# Autodesk Inventor assembly: roka
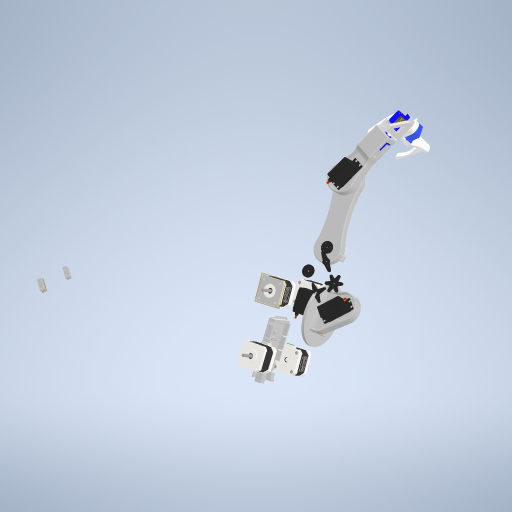
[picture p0: Inventor's stored thumbnail of the model, 512x512]
Saved by Autodesk Inventor 2024 (Build 280153000, 153)
## iProperties
Created: 2023-09-17
Part Number: roka
Document SubType Name: Assembly
Designer: jebes windows
Author: jebes windows
## Documents named in this file (13)
- C:\Users\jebes windows\Documents\Inventor\Robotska_roka\roka.iam
- C:\Users\jebes windows\Documents\Inventor\Robotska_roka\Nema 17 Motor a Pasos 17HS4401\Nema 17 Motor a Pasos 17HS4401.ipt
- C:\Users\jebes windows\Documents\Inventor\Robotska_roka\ArduinoMega_STEP_AP203\ArduinoMega_STEP_AP203.ipt
- C:\Users\jebes windows\Documents\Inventor\Robotska_roka\servo-motor-mg996r-1.snapshot.1(2)\Servo Motor MG996R  With Attachments\Servo Motor MG996R  With Attachments.iam
- C:\Users\jebes windows\Documents\Inventor\Robotska_roka\miza.ipt
- C:\Users\jebes windows\Documents\Inventor\Robotska_roka\roka1.ipt
- C:\Users\jebes windows\Documents\Inventor\Robotska_roka\roka2.ipt
- C:\Users\jebes windows\Documents\Inventor\Robotska_roka\sg90-micro-servo-9g-tower-pro-1.snapshot.3\SG90 - Micro Servo 9g - Tower Pro\SG90 - Micro Servo 9g - Tower Pro.iam
- C:\Users\jebes windows\Documents\Inventor\Robotska_roka\roka3.ipt
- C:\Users\jebes windows\Documents\Inventor\Robotska_roka\linear-gripper-1.snapshot.4\Linear Gripper\GRIPPER.iam
- C:\Users\jebes windows\Documents\Inventor\Robotska_roka\Part2.ipt
- C:\Users\jebes windows\Documents\Inventor\Robotska_roka\buh.ipt
- C:\Users\jebes windows\Documents\Inventor\Robotska_roka\buh2.ipt
## Components (22 placed, 12 different names)
1. Nema 17 Motor a Pasos 17HS4401:1
2. Nema 17 Motor a Pasos 17HS4401:2
3. Nema 17 Motor a Pasos 17HS4401:3 — Flush:1, Flush:2
4. Nema 17 Motor a Pasos 17HS4401:4
5. ArduinoMega_STEP_AP203:1
6. Servo Motor MG996R  With Attachments:1 [sub-assembly] — Rotational:1
7. Servo Motor MG996R  With Attachments:2 [sub-assembly] — Rotational:1, Rigid:7
8. miza:1 — Rigid:7
9. Servo Motor MG996R  With Attachments:3 [sub-assembly]
10. Servo Motor MG996R  With Attachments:4 [sub-assembly] — Rotational:3, Angle:1
11. roka1:1 — Rotational:3, Rotational:5
12. roka2:1 — Rigid:10, Rigid:11
13. Servo Motor MG996R  With Attachments:5 [sub-assembly] — Rigid:10
14. Servo Motor MG996R  With Attachments:6 [sub-assembly] — Rotational:5
15. SG90 - Micro Servo 9g - Tower Pro:1 [sub-assembly] — Rigid:11, Rotational:6
16. SG90 - Micro Servo 9g - Tower Pro:3 [sub-assembly] — Rigid:13, Rotational:12
17. roka3:1 — Rigid:13, Rotational:6
18. GRIPPER:1 [sub-assembly] — Rotational:12
19. Part2:1 — Flush:1, Flush:2
20. Servo Motor MG996R  With Attachments:7 [sub-assembly] — Flush:3, Flush:4, Flush:5, Flush:6
21. buh:1 — Flush:3, Flush:4
22. buh2:1 — Flush:5, Flush:6
## Relationships (17: RevoluteJoint 6, Flush 6, WeldJoint 4, Angle 1)
- Rotational:1 [RevoluteJoint]: Servo Motor MG996R  With Attachments:1 ↔ Servo Motor MG996R  With Attachments:2
- Rigid:7 [WeldJoint]: Servo Motor MG996R  With Attachments:2 ↔ miza:1
- Rotational:3 [RevoluteJoint]: Servo Motor MG996R  With Attachments:4 ↔ roka1:1
- [RevoluteJoint]: Servo Motor MG996R  With Attachments:5 ↔ Servo Motor MG996R  With Attachments:6
- Rigid:10 [WeldJoint]: roka2:1 ↔ Servo Motor MG996R  With Attachments:5
- Rotational:5 [RevoluteJoint]: roka1:1 ↔ Servo Motor MG996R  With Attachments:6
- Rigid:11 [WeldJoint]: roka2:1 ↔ SG90 - Micro Servo 9g - Tower Pro:1
- Rigid:13 [WeldJoint]: SG90 - Micro Servo 9g - Tower Pro:3 ↔ roka3:1
- Rotational:6 [RevoluteJoint]: SG90 - Micro Servo 9g - Tower Pro:1 ↔ roka3:1
- Angle:1 (0 deg): Servo Motor MG996R  With Attachments:4
- Rotational:12 [RevoluteJoint]: SG90 - Micro Servo 9g - Tower Pro:3 ↔ GRIPPER:1
- Flush:1: Nema 17 Motor a Pasos 17HS4401:3 ↔ Part2:1
- Flush:2: Nema 17 Motor a Pasos 17HS4401:3 ↔ Part2:1
- Flush:3: Servo Motor MG996R  With Attachments:7 ↔ buh:1
- Flush:4: Servo Motor MG996R  With Attachments:7 ↔ buh:1
- Flush:5: Servo Motor MG996R  With Attachments:7 ↔ buh2:1
- Flush:6: Servo Motor MG996R  With Attachments:7 ↔ buh2:1
## Named parameters: d15_d11 = 0 mm, d16_d12 = 64.240964 deg
